# Autodesk Inventor assembly: DB_DriveBase_Long Pneumatic Wheels
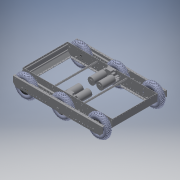
[picture p0: Inventor's stored thumbnail of the model, 180x180]
Saved by Autodesk Inventor 2016 (Build 200138000, 138)
## iProperties
Created: 2014-01-06
Part Number: DB_DriveBase_Long Pneumatic Wheels
Document SubType Name: Assembly
Designer: Robotics-04
Title: C:\Users\Philip\Desktop\FIRST Drive Base Long\STEP\DB_DriveBase_Long.stp
Author: Philip
Sending System: Autodesk Inventor 2014
Preprocessor: ST-DEVELOPER v15.2
## Documents named in this file (3)
- C:\Users\Robotics-04\Desktop\JACOB NO TOUCHY\DB_DriveBase_Long Pneumatic Wheels.iam
- C:\Users\Robotics-04\Desktop\JACOB NO TOUCHY\AM14U Long.iam
- C:\Users\Robotics-04\Desktop\Wheels\PneumaticWheel_am-0970 (3).iam
## Components (7 placed, 2 different names)
1. AM14U Long_2 [sub-assembly] — Rigid:1, Rigid:2, Rotational:1, Rigid:3, Rigid:4, Rotational:2
2. PneumaticWheel_am-0970 (3):1 [sub-assembly] — Rotational:2
3. PneumaticWheel_am-0970 (3):2 [sub-assembly] — Rigid:1
4. PneumaticWheel_am-0970 (3):3 [sub-assembly] — Rigid:2
5. PneumaticWheel_am-0970 (3):4 [sub-assembly] — Rigid:3
6. PneumaticWheel_am-0970 (3):5 [sub-assembly] — Rotational:1
7. PneumaticWheel_am-0970 (3):6 [sub-assembly] — Rigid:4
## Relationships (6: WeldJoint 4, RevoluteJoint 2)
- Rigid:1 [WeldJoint] (-60.325 mm): AM14U Long_2 ↔ PneumaticWheel_am-0970 (3):2
- Rigid:2 [WeldJoint] (-71.4375 mm): AM14U Long_2 ↔ PneumaticWheel_am-0970 (3):3
- Rotational:1 [RevoluteJoint] (-41.275 mm): AM14U Long_2 ↔ PneumaticWheel_am-0970 (3):5
- Rigid:3 [WeldJoint] (-33.3375 mm): AM14U Long_2 ↔ PneumaticWheel_am-0970 (3):4
- Rigid:4 [WeldJoint] (-66.675 mm): AM14U Long_2 ↔ PneumaticWheel_am-0970 (3):6
- Rotational:2 [RevoluteJoint] (-36.5125 mm): AM14U Long_2 ↔ PneumaticWheel_am-0970 (3):1
